# Autodesk Inventor assembly: T1
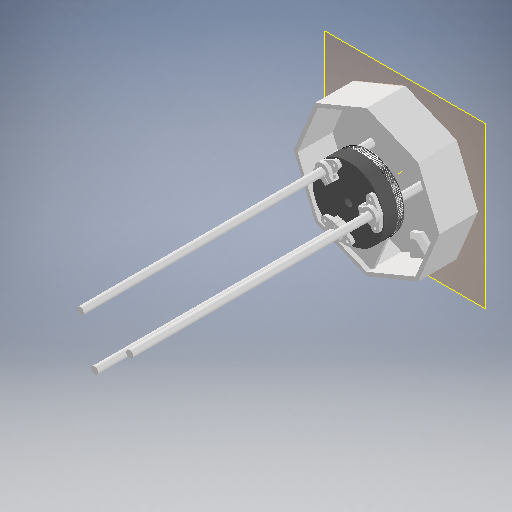
[picture p0: Inventor's stored thumbnail of the model, 512x512]
Saved by Autodesk Inventor 2025.2 (Build 292293000, 293)
## iProperties
Created: 2025-04-07
Part Number: T1
Document SubType Name: Assembly
Designer: Tiago
Author: Tiago
## Documents named in this file (9)
- C:\Users\Tiago\Documents\Inventor\Exp. Braço v1\T1.iam
- C:\Users\Tiago\Documents\Inventor\Exp. Braço v1\BaseHex.ipt
- C:\Users\Tiago\Documents\Inventor\Exp. Braço v1\NEMA17 42-38.ipt
- C:\Users\Tiago\Documents\Inventor\Exp. Braço v1\Base_Chanf.ipt
- C:\Users\Tiago\Documents\Inventor\Exp. Braço v1\Nem_pulley.ipt
- C:\Users\Tiago\Documents\Inventor\Exp. Braço v1\Big_pulley.ipt
- C:\Users\Tiago\Documents\Inventor\Exp. Braço v1\Base_Junta.ipt
- C:\Users\Tiago\Documents\Inventor\Exp. Braço v1\Linear_Shaft_Support_SHF10.ipt
- C:\Users\Tiago\Documents\Inventor\Exp. Braço v1\rodshaft_10x400.ipt
## Components (12 placed, 8 different names)
1. BaseHex:1 — Mate:1, Mate:2, Mate:3, Mate:4, Mate:6, Flush:1, Flush:2, Mate:9, Mate:10
2. NEMA17 42-38:1 — Mate:3, Mate:4, Mate:7
3. Base_Chanf:1 — Mate:6, Mate:9, Mate:10
4. Synchronous Pulley1:1 — Mate:7, Flush:1
5. Synchronous Pulley2:1 — Mate:8, Flush:2, Mate:12
6. Base_Junta:1 — Mate:11, Mate:12, Mate:13, Mate:14, Mate:15, Mate:16, Mate:17, Mate:18, Mate:19, Mate:20, Mate:21
7. Linear_Shaft_Support_SHF10:1 — Mate:15, Mate:16, Mate:20, Mate:23
8. Linear_Shaft_Support_SHF10:2 — Mate:14, Mate:18, Mate:21, Mate:24
9. Linear_Shaft_Support_SHF10:3 — Mate:13, Mate:17, Mate:19, Mate:22
10. rodshaft_10x400:1 — Mate:22
11. rodshaft_10x400:2 — Mate:23
12. rodshaft_10x400:3 — Mate:24
## Relationships (25: Mate 23, Flush 2)
- Mate:1: BaseHex:1
- Mate:2: BaseHex:1
- Mate:3: BaseHex:1 ↔ NEMA17 42-38:1
- Mate:4: BaseHex:1 ↔ NEMA17 42-38:1
- Mate:6: BaseHex:1 ↔ Base_Chanf:1
- Mate:7: NEMA17 42-38:1 ↔ Synchronous Pulley1:1
- Flush:1 (-12 mm): BaseHex:1 ↔ Synchronous Pulley1:1
- Mate:8: Synchronous Pulley2:1
- Flush:2 (12 mm): BaseHex:1 ↔ Synchronous Pulley2:1
- Mate:9: BaseHex:1 ↔ Base_Chanf:1
- Mate:10: BaseHex:1 ↔ Base_Chanf:1
- Mate:11: Base_Junta:1
- Mate:12: Synchronous Pulley2:1 ↔ Base_Junta:1
- Mate:13: Base_Junta:1 ↔ Linear_Shaft_Support_SHF10:3
- Mate:14: Base_Junta:1 ↔ Linear_Shaft_Support_SHF10:2
- Mate:15: Base_Junta:1 ↔ Linear_Shaft_Support_SHF10:1
- Mate:16: Base_Junta:1 ↔ Linear_Shaft_Support_SHF10:1
- Mate:17: Base_Junta:1 ↔ Linear_Shaft_Support_SHF10:3
- Mate:18: Base_Junta:1 ↔ Linear_Shaft_Support_SHF10:2
- Mate:19: Base_Junta:1 ↔ Linear_Shaft_Support_SHF10:3
- Mate:20: Base_Junta:1 ↔ Linear_Shaft_Support_SHF10:1
- Mate:21: Base_Junta:1 ↔ Linear_Shaft_Support_SHF10:2
- Mate:22: Linear_Shaft_Support_SHF10:3 ↔ rodshaft_10x400:1
- Mate:23: Linear_Shaft_Support_SHF10:1 ↔ rodshaft_10x400:2
- Mate:24: Linear_Shaft_Support_SHF10:2 ↔ rodshaft_10x400:3
